# Autodesk Inventor assembly: 130
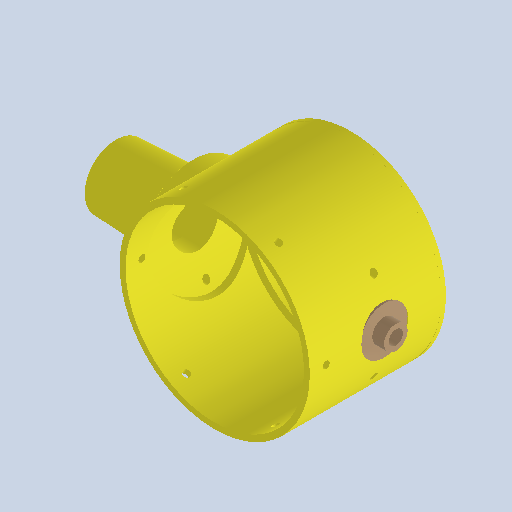
[picture p0: Inventor's stored thumbnail of the model, 512x512]
Saved by Autodesk Inventor 2025.1 (Build 291241000, 241)
## iProperties
Created: 2024-08-01
Part Number: 130
Document SubType Name: Assembly
Designer: ffogue
Author: ffogue
## Documents named in this file (5)
- C:\Projkete - Übungen\Freedom\130.iam
- C:\Projkete - Übungen\Freedom\130 part 3.ipt
- C:\Projkete - Übungen\Freedom\130 part 1.ipt
- C:\Projkete - Übungen\Freedom\130 part 2.ipt
- C:\Projkete - Übungen\Freedom\131.ipt
## Components (4 placed, 4 different names)
1. 130 part 1:1 — Rotational:1, Insert:1, Rotational:2
2. 130 part 3:1 — Rotational:1
3. 130 part 2:1 — Insert:1
4. 131:1 — Rotational:2
## Relationships (3: RevoluteJoint 2, Insert 1)
- Rotational:1 [RevoluteJoint] (-0.5 mm): 130 part 1:1 ↔ 130 part 3:1
- Insert:1: 130 part 1:1 ↔ 130 part 2:1
- Rotational:2 [RevoluteJoint] (-7 mm): 130 part 1:1 ↔ 131:1
